# Autodesk Inventor assembly: LedPlane
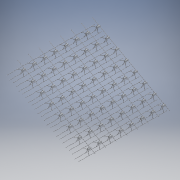
[picture p0: Inventor's stored thumbnail of the model, 180x180]
Saved by Autodesk Inventor 2019.3 (Build 233278000, 278)
## iProperties
Created: 2019-01-09
Part Number: LedPlane
Material: Generisch
Document SubType Name: Assembly
Designer: Jonas
Author: Jonas
## Documents named in this file (3)
- C:\Users\Jonas\Desktop\RGBCube\RGBCubev2\CAD\Led\LedPlane.iam
- C:\Users\Jonas\Desktop\RGBCube\RGBCubev2\CAD\Led\LedRow.iam
- C:\Users\Jonas\Desktop\RGBCube\RGBCubev2\CAD\Led\WireAnode.ipt
## Components (32 placed, 2 different names)
1. LedRow:1 [sub-assembly] — Einfügen:1, Passend:13, Passend:14, Einfügen:11
2. LedRow:2 [sub-assembly] — Einfügen:2, Passend:11, Passend:12, Einfügen:12, Einfügen:13
3. LedRow:3 [sub-assembly] — Einfügen:3, Passend:9, Passend:10, Einfügen:14
4. LedRow:4 [sub-assembly] — Einfügen:4, Passend:7, Passend:8, Einfügen:15
5. LedRow:5 [sub-assembly] — Einfügen:5, Passend:5, Passend:6
6. LedRow:6 [sub-assembly] — Einfügen:6, Passend:3, Passend:4
7. LedRow:7 [sub-assembly] — Einfügen:7, Passend:1, Passend:2
8. LedRow:8 [sub-assembly] — Einfügen:8, Einfügen:9, Einfügen:10, Einfügen:16, Einfügen:17, Einfügen:18, Einfügen:19, Einfügen:20, Einfügen:21, Einfügen:22, Einfügen:23, Einfügen:24, Einfügen:25, Einfügen:26, Einfügen:27, Einfügen:28, Einfügen:29, Einfügen:30, Einfügen:31, Einfügen:32, Einfügen:33, Einfügen:34, Einfügen:35
9. WireAnode:1 — Einfügen:1, Einfügen:2, Einfügen:3, Einfügen:4, Einfügen:5, Einfügen:6, Einfügen:7, Einfügen:8
10. WireAnode:2 — Einfügen:9, Passend:1, Passend:3, Passend:5, Passend:7, Passend:9, Passend:11, Passend:13
11. WireAnode:3 — Einfügen:10, Passend:2, Passend:4, Passend:6, Passend:8, Passend:10, Passend:12, Passend:14
12. WireAnode:4 — Einfügen:11, Einfügen:12, Einfügen:13, Einfügen:14, Einfügen:15
13. WireAnode:5 — Einfügen:16
14. WireAnode:6 — Einfügen:17
15. WireAnode:7 — Einfügen:18
16. WireAnode:8 — Einfügen:20
17. WireAnode:9 — Einfügen:19
18. WireAnode:10 — Einfügen:24
19. WireAnode:11 — Einfügen:26
20. WireAnode:12 — Einfügen:25
21. WireAnode:13 — Einfügen:27
22. WireAnode:14 — Einfügen:28
23. WireAnode:15 — Einfügen:29
24. WireAnode:16 — Einfügen:21
25. WireAnode:17 — Einfügen:22
26. WireAnode:18 — Einfügen:23
27. WireAnode:19 — Einfügen:35
28. WireAnode:20 — Einfügen:34
29. WireAnode:21 — Einfügen:33
30. WireAnode:22 — Einfügen:32
31. WireAnode:23 — Einfügen:31
32. WireAnode:24 — Einfügen:30
## Relationships (49: Insert 35, Mate 14)
- Einfügen:1 [Insert] (-10 mm): LedRow:1 ↔ WireAnode:1
- Einfügen:2 [Insert] (-40 mm): LedRow:2 ↔ WireAnode:1
- Einfügen:3 [Insert] (-70 mm): LedRow:3 ↔ WireAnode:1
- Einfügen:4 [Insert] (-100 mm): LedRow:4 ↔ WireAnode:1
- Einfügen:5 [Insert] (-130 mm): LedRow:5 ↔ WireAnode:1
- Einfügen:6 [Insert] (-160 mm): LedRow:6 ↔ WireAnode:1
- Einfügen:7 [Insert] (-190 mm): LedRow:7 ↔ WireAnode:1
- Einfügen:8 [Insert] (-220 mm): LedRow:8 ↔ WireAnode:1
- Einfügen:9 [Insert] (-220 mm): LedRow:8 ↔ WireAnode:2
- Einfügen:10 [Insert] (-220 mm): LedRow:8 ↔ WireAnode:3
- Passend:1 [Mate]: LedRow:7 ↔ WireAnode:2
- Passend:2 [Mate]: LedRow:7 ↔ WireAnode:3
- Passend:3 [Mate]: LedRow:6 ↔ WireAnode:2
- Passend:4 [Mate]: LedRow:6 ↔ WireAnode:3
- Passend:5 [Mate]: LedRow:5 ↔ WireAnode:2
- Passend:6 [Mate]: LedRow:5 ↔ WireAnode:3
- Passend:7 [Mate]: LedRow:4 ↔ WireAnode:2
- Passend:8 [Mate]: LedRow:4 ↔ WireAnode:3
- Passend:9 [Mate]: LedRow:3 ↔ WireAnode:2
- Passend:10 [Mate]: LedRow:3 ↔ WireAnode:3
- Passend:11 [Mate]: LedRow:2 ↔ WireAnode:2
- Passend:12 [Mate]: LedRow:2 ↔ WireAnode:3
- Passend:13 [Mate]: LedRow:1 ↔ WireAnode:2
- Passend:14 [Mate]: LedRow:1 ↔ WireAnode:3
- Einfügen:11 [Insert] (-10 mm): LedRow:1 ↔ WireAnode:4
- Einfügen:12 [Insert] (-40 mm): LedRow:2 ↔ WireAnode:4
- Einfügen:13 [Insert] (-40 mm): LedRow:2 ↔ WireAnode:4
- Einfügen:14 [Insert] (-70 mm): LedRow:3 ↔ WireAnode:4
- Einfügen:15 [Insert] (-100 mm): LedRow:4 ↔ WireAnode:4
- Einfügen:16 [Insert] (-220 mm): LedRow:8 ↔ WireAnode:5
- Einfügen:17 [Insert] (-220 mm): LedRow:8 ↔ WireAnode:6
- Einfügen:18 [Insert] (-220 mm): LedRow:8 ↔ WireAnode:7
- Einfügen:19 [Insert] (-220 mm): LedRow:8 ↔ WireAnode:9
- Einfügen:20 [Insert] (-220 mm): LedRow:8 ↔ WireAnode:8
- Einfügen:21 [Insert] (-220 mm): LedRow:8 ↔ WireAnode:16
- Einfügen:22 [Insert] (-220 mm): LedRow:8 ↔ WireAnode:17
- Einfügen:23 [Insert] (-220 mm): LedRow:8 ↔ WireAnode:18
- Einfügen:24 [Insert] (-220 mm): LedRow:8 ↔ WireAnode:10
- Einfügen:25 [Insert] (-220 mm): LedRow:8 ↔ WireAnode:12
- Einfügen:26 [Insert] (-220 mm): LedRow:8 ↔ WireAnode:11
- Einfügen:27 [Insert] (-220 mm): LedRow:8 ↔ WireAnode:13
- Einfügen:28 [Insert] (-220 mm): LedRow:8 ↔ WireAnode:14
- Einfügen:29 [Insert] (-220 mm): LedRow:8 ↔ WireAnode:15
- Einfügen:30 [Insert] (-220 mm): LedRow:8 ↔ WireAnode:24
- Einfügen:31 [Insert] (-220 mm): LedRow:8 ↔ WireAnode:23
- Einfügen:32 [Insert] (-220 mm): LedRow:8 ↔ WireAnode:22
- Einfügen:33 [Insert] (-220 mm): LedRow:8 ↔ WireAnode:21
- Einfügen:34 [Insert] (-220 mm): LedRow:8 ↔ WireAnode:20
- Einfügen:35 [Insert] (-220 mm): LedRow:8 ↔ WireAnode:19
